# Autodesk Inventor assembly: Z
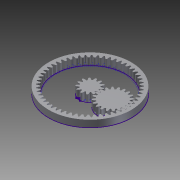
[picture p0: Inventor's stored thumbnail of the model, 180x180]
Saved by Autodesk Inventor 2014 (Build 180170000, 170)
## iProperties
Created: 2013-05-24
Part Number: Z
Document SubType Name: Assembly
Designer: hartmann
Author: hartmann
## Documents named in this file (4)
- C:\Dokumente und Einstellungen\hartmann\Desktop\Z132053\Z.iam
- C:\Dokumente und Einstellungen\hartmann\Desktop\Z132053\Z13.ipt
- C:\Dokumente und Einstellungen\hartmann\Desktop\Z132053\Z20.ipt
- C:\Dokumente und Einstellungen\hartmann\Desktop\Z132053\Z53.ipt
## Components (3 placed, 3 different names)
1. Z13:1 — Passend:1, Fluchtend:1, Passend:4, Drehung:2
2. Z20:1 — Passend:3, Fluchtend:1, Fluchtend:2, Drehung:1, Drehung:2
3. Z53:1 — Passend:2, Fluchtend:2, Drehung:1
## Relationships (8: Mate 4, Flush 2, RelateRotation 2)
- Passend:1 [Mate]: Z13:1
- Passend:2 [Mate]: Z53:1
- Passend:3 [Mate] (6.647 mm): Z20:1
- Fluchtend:1 [Flush]: Z13:1 ↔ Z20:1
- Fluchtend:2 [Flush]: Z20:1 ↔ Z53:1
- Passend:4 [Mate]: Z13:1
- Drehung:1 [RelateRotation] (2.65 ul): Z20:1 ↔ Z53:1
- Drehung:2 [RelateRotation] (1.5 ul): Z13:1 ↔ Z20:1
